# Autodesk Inventor assembly: Sharp GP2Y0 Sensor
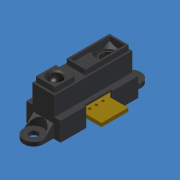
[picture p0: Inventor's stored thumbnail of the model, 180x180]
Saved by Autodesk Inventor 2012 (Build 160160000, 160)
## iProperties
Category: FIRST
Manager: Ed Sparks
Company: FirstCadLibrary
Shininess: 64.0
Length Units: 11272
Angle Units: 11279
Time Units: 11290
Mass Units: 11286
Length Display Precision: 3
Angle Display Precision: 2
Compacted: True
Part Number: Sharp GP2Y0 Sensor
Document SubType Name: Assembly
Created: 2007-12-20
Designer: Owner
Project: FIRST
Catalog Web Link: www.firstcadlibrary.com
Engineer: Ed Sparks
Mass: 2.09892 g
Surface Area: 43.1665 cm^2
Volume: 1.83553 cm^3
Density: 1.14349 g/cm^3
Density: 0.0
Volumn: 0.0
Area: 0.0
PropertySet Name: Model Information
Control State: 0
Master: False
Checked Out: False
Author: Owner
Keywords: FIRST
## Documents named in this file (3)
- C:\Users\Admin\Documents\Inventor\SumoJaime2012\Sharp GP2Y0 Sensor.iam
- C:\Users\Admin\Documents\Inventor\SumoJaime2012\Sharp GP2Y0 Sensor Housing.ipt
- C:\Users\Admin\Documents\Inventor\SumoJaime2012\Sharp GP2Y0 Sensor PCB.ipt
## Components (2 placed, 2 different names)
1. Sharp GP2Y0 Sensor Housing:1 — Mate:1, Flush:1, Flush:2
2. Sharp GP2Y0 Sensor PCB:1 — Mate:1, Flush:1, Flush:2
## Relationships (3: Flush 2, Mate 1)
- Mate:1: Sharp GP2Y0 Sensor Housing:1 ↔ Sharp GP2Y0 Sensor PCB:1
- Flush:1: Sharp GP2Y0 Sensor Housing:1 ↔ Sharp GP2Y0 Sensor PCB:1
- Flush:2 (3.25 mm): Sharp GP2Y0 Sensor Housing:1 ↔ Sharp GP2Y0 Sensor PCB:1
